# Autodesk Inventor assembly: Assembly1
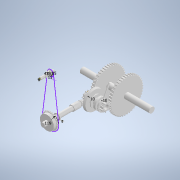
[picture p0: Inventor's stored thumbnail of the model, 180x180]
Saved by Autodesk Inventor 2021 (Build 250183000, 183)
## iProperties
Created: 2022-12-13
Part Number: Assembly1
Document SubType Name: Assembly
Designer: user
Author: user
## Documents named in this file (17)
- C:\Users\user\Desktop\Major\Assembly1.iam
- C:\Users\user\Desktop\Major\Part1.ipt
- C:\Users\user\Desktop\Major\Part2.ipt
- C:\Users\user\Desktop\Major\Part4.ipt
- C:\Users\user\Desktop\Major\Part5.ipt
- C:\Users\user\Desktop\Major\part6.ipt
- C:\Users\user\Desktop\Major\part7.ipt
- C:\Users\user\Desktop\Major\part8.ipt
- C:\Users\user\Desktop\Major\Part9.ipt
- C:\Users\user\Desktop\Major\Part10.ipt
- C:\Users\user\Desktop\Major\Part11.ipt
- C:\Users\user\Desktop\Major\Part12.ipt
- C:\Users\user\Desktop\Major\Part13.ipt
- C:\Users\user\Desktop\Major\Part14.ipt
- C:\Users\user\Desktop\Major\Part15.ipt
- C:\Users\user\Documents\Inventor\Content Center Files\R2021\en-US\ISO 7380-1\ISO 7380-1 - M8 x 10.ipt
- C:\Users\user\Documents\Inventor\Content Center Files\R2021\en-US\ISO 7380-1\ISO 7380-1 - M6 x 10.ipt
## Components (21 placed, 16 different names)
1. Part1:1 — Mate:1, Mate:3, Mate:4, Flush:6
2. Part2:1 — Mate:2, Mate:3, Mate:4, Flush:2, Flush:3
3. Part4:1 — Flush:3, Mate:5, Flush:5, Mate:6, Mate:7, Flush:7, Mate:28
4. Part5:1 — Mate:7, Flush:7, Mate:8, Mate:9, Mate:12, Mate:13, Mate:14, Mate:15
5. DIN 625 SKF SKF 61806:1 — Mate:8, Mate:10, Flush:8
6. part7:1 — Mate:9, Mate:10, Flush:9, Flush:13, Mate:42, Mate:43, Mate:44, Mate:45
7. part8:1 — Mate:12, Mate:13, Mate:14, Flush:14
8. Part9:1 — Mate:15, Mate:16, Mate:19, Mate:29, Mate:33, Mate:37, Mate:38
9. Part10:1 — Mate:29, Mate:30, Mate:32, Mate:34, Mate:37
10. Part11:1 — Mate:22, Mate:30, Mate:31, Mate:32, Mate:34, Mate:35, Mate:41
11. Part11:2 — Mate:19, Mate:21, Mate:23, Mate:27, Mate:36, Mate:38, Mate:40
12. Part12:1 — Mate:22
13. Part12:2 — Mate:21
14. Part13:1 — Mate:31, Mate:35
15. Part13:2 — Mate:27, Mate:36
16. Part14:1 — Mate:25, Mate:41
17. Part14:2 — Mate:24, Mate:40
18. Part15:1 — Mate:23, Mate:24, Mate:25, Angle:1, Mate:39
19. ISO 7380-1 M6 x 10:1 — Mate:42, Mate:45
20. ISO 7380-1 M8 x 10:2
21. ISO 7380-1 M6 x 10:2 — Mate:43, Mate:44
## Relationships (52: Mate 41, Flush 10, Angle 1)
- Mate:1: Part1:1
- Mate:2: Part2:1
- Mate:3: Part1:1 ↔ Part2:1
- Mate:4 (80 mm): Part1:1 ↔ Part2:1
- Flush:2 (-3 mm): Part2:1
- Flush:3: Part2:1 ↔ Part4:1
- Flush:4 (-300 mm)
- Mate:5: Part4:1
- Flush:5 (-5 mm): Part4:1
- Flush:6 (6.673 mm): Part1:1
- Mate:6: Part4:1
- Mate:7: Part4:1 ↔ Part5:1
- Flush:7 (200 mm): Part4:1 ↔ Part5:1
- Mate:8: Part5:1 ↔ DIN 625 SKF SKF 61806:1
- Mate:9: Part5:1 ↔ part7:1
- Mate:10: DIN 625 SKF SKF 61806:1 ↔ part7:1
- Flush:8 (-3.5 mm): DIN 625 SKF SKF 61806:1
- Flush:9 (-4 mm): part7:1
- Mate:11
- Flush:13: part7:1
- Mate:12: Part5:1 ↔ part8:1
- Mate:13: Part5:1 ↔ part8:1
- Mate:14: Part5:1 ↔ part8:1
- Mate:15: Part5:1 ↔ Part9:1
- Mate:16 (21 mm): Part9:1
- Mate:19: Part9:1 ↔ Part11:2
- Mate:21: Part11:2 ↔ Part12:2
- Mate:22: Part11:1 ↔ Part12:1
- Mate:23 (147 mm): Part11:2 ↔ Part15:1
- Mate:24: Part14:2 ↔ Part15:1
- Mate:25: Part14:1 ↔ Part15:1
- Mate:27: Part11:2 ↔ Part13:2
- Mate:28: Part4:1
- Mate:29: Part9:1 ↔ Part10:1
- Mate:30: Part10:1 ↔ Part11:1
- Mate:31: Part11:1 ↔ Part13:1
- Mate:32: Part10:1 ↔ Part11:1
- Flush:14 (50 mm): part8:1
- Mate:33: Part9:1
- Mate:34: Part10:1 ↔ Part11:1
- Mate:35: Part11:1 ↔ Part13:1
- Mate:36: Part11:2 ↔ Part13:2
- Mate:37 (5 mm): Part9:1 ↔ Part10:1
- Mate:38: Part9:1 ↔ Part11:2
- Angle:1 (0 deg): Part15:1
- Mate:39 (-515.67 mm): Part15:1
- Mate:40: Part11:2 ↔ Part14:2
- Mate:41: Part11:1 ↔ Part14:1
- Mate:42: part7:1 ↔ ISO 7380-1 M6 x 10:1
- Mate:43: part7:1 ↔ ISO 7380-1 M6 x 10:2
- Mate:44: part7:1 ↔ ISO 7380-1 M6 x 10:2
- Mate:45: part7:1 ↔ ISO 7380-1 M6 x 10:1
